# Autodesk Inventor assembly: Quadropod_assembly_v2
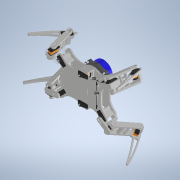
[picture p0: Inventor's stored thumbnail of the model, 180x180]
Saved by Autodesk Inventor 2020.3 (Build 243373000, 373)
## iProperties
Created: 2021-03-19
Part Number: Quadropod_assembly_v2
Document SubType Name: Assembly
Designer: sanyi
Author: sanyi
## Documents named in this file (15)
- C:\Users\sanyi\Documents\Inventor\Quadropod\Quadropod_assembly_v2.iam
- C:\Users\sanyi\Documents\Inventor\Quadropod\BaseBottom_v1.ipt
- C:\Users\sanyi\Documents\Inventor\Quadropod\LegPin_Middle_v1.ipt
- C:\Users\sanyi\Documents\Inventor\Quadropod\LegPin_Side_v1.ipt
- C:\Users\sanyi\Documents\Inventor\Quadropod\LegPin_Side_v1_MIR.ipt
- C:\Users\sanyi\Documents\Inventor\Quadropod\BaseTop_v1.ipt
- C:\Users\sanyi\Documents\Inventor\Quadropod\SH-0257MG.ipt
- C:\Users\sanyi\Documents\Inventor\Quadropod\LegStart_v1.ipt
- C:\Users\sanyi\Documents\Inventor\Quadropod\LegStart_v1_MIR.ipt
- C:\Users\sanyi\Documents\Inventor\Quadropod\ydlidar x4.ipt
- C:\Users\sanyi\Documents\Inventor\Quadropod\LegPin_v1.ipt
- C:\Users\sanyi\Documents\Inventor\Quadropod\LegMiddle_Final_1.ipt
- C:\Users\sanyi\Documents\Inventor\Quadropod\LegEnd_Right_v1.ipt
- C:\Users\sanyi\Documents\Inventor\Quadropod\LegEnd_Right_v1_MIR.ipt
- C:\Users\sanyi\Documents\Inventor\Quadropod\LegEnd_Right_v2.ipt
## Components (43 placed, 14 different names)
1. BaseBottom_v1:1 — Insert:1, Insert:2, Insert:3, Insert:4, Insert:5, Insert:6, Insert:7, Insert:8, Flush:1, Flush:2, Mate:1, Insert:9, Insert:10, Insert:11, Insert:12, Insert:15, Angle:1, Angle:2, Insert:16, Insert:17, Insert:18, Insert:19, Insert:20, Angle:3, Angle:4, Angle:5, Angle:6
2. LegPin_Middle_v1:1 — Insert:1, Insert:2
3. LegPin_Middle_v1:2 — Insert:3, Insert:4, Insert:13, Mate:2
4. LegPin_Middle_v1:3 — Insert:5, Insert:6
5. LegPin_Middle_v1:4 — Insert:7, Insert:8, Insert:14
6. LegPin_Side_v1:1 — Insert:9, Insert:10
7. LegPin_Side_v1_MIR:1 — Insert:11, Insert:12
8. BaseTop_v1:1 — Insert:13, Insert:14, Mate:2, Insert:59, Insert:60
9. SH-0257MG:1 — Insert:15, Angle:1, Insert:22
10. SH-0257MG:2 — Angle:2, Insert:16, Insert:23
11. SH-0257MG:3 — Insert:17, Angle:3
12. SH-0257MG:4 — Insert:20, Angle:6
13. SH-0257MG:5 — Insert:19, Angle:5, Insert:21
14. SH-0257MG:6 — Insert:18, Angle:4, Insert:24
15. LegStart_v1:2 — Insert:21, Insert:27, Angle:7, Insert:35, Insert:36
16. LegStart_v1:3 — Insert:23, Insert:30, Angle:10, Insert:31, Insert:32
17. LegStart_v1_MIR:1 — Insert:24, Insert:29, Angle:9, Insert:33, Insert:34
18. LegStart_v1_MIR:2 — Insert:22, Insert:28, Angle:8, Insert:37, Insert:38
19. ydlidar x4:1 — Flush:3, Insert:59, Insert:60
20. SH-0257MG:7 — Insert:27, Angle:7, Insert:41
21. SH-0257MG:8 — Insert:29, Angle:9, Insert:42
22. SH-0257MG:9 — Insert:28, Angle:8, Insert:39
23. SH-0257MG:10 — Insert:30, Angle:10, Insert:40
24. SH-0257MG:11 — Insert:55, Angle:15, Insert:63
25. SH-0257MG:12 — Insert:44, Angle:12, Insert:57
26. SH-0257MG:13 — Insert:45, Angle:13, Insert:58
27. SH-0257MG:14 — Insert:46, Angle:14, Insert:56
28. LegPin_v1:1 — Insert:31, Insert:32
29. LegPin_v1:2 — Insert:33, Insert:34
30. LegPin_v1:3 — Insert:37, Insert:38
31. LegPin_v1:4 — Insert:61, Insert:62
32. LegPin_v1:5 — Insert:49, Insert:50
33. LegPin_v1:6 — Insert:51, Insert:52
34. LegPin_v1:7 — Insert:53, Insert:54
35. LegPin_v1:8 — Insert:35, Insert:36
36. LegMiddle_Final_1:1 — Insert:39, Insert:56
37. LegMiddle_Final_1:2 — Insert:40, Insert:55
38. LegMiddle_Final_1:3 — Insert:42, Insert:58
39. LegMiddle_Final_1:4 — Insert:41, Insert:57
40. LegEnd_Right_v1:2 — Insert:44, Angle:12, Insert:49, Insert:50
41. LegEnd_Right_v1_MIR:1 — Insert:45, Angle:13, Insert:51, Insert:52
42. LegEnd_Right_v1_MIR:2 — Insert:46, Angle:14, Insert:53, Insert:54
43. LegEnd_Right_v2:1 — Angle:15, Insert:61, Insert:62, Insert:63
## Relationships (77: Insert 58, Angle 14, Flush 3, Mate 2)
- Insert:1: BaseBottom_v1:1 ↔ LegPin_Middle_v1:1
- Insert:2: BaseBottom_v1:1 ↔ LegPin_Middle_v1:1
- Insert:3: BaseBottom_v1:1 ↔ LegPin_Middle_v1:2
- Insert:4: BaseBottom_v1:1 ↔ LegPin_Middle_v1:2
- Insert:5: BaseBottom_v1:1 ↔ LegPin_Middle_v1:3
- Insert:6: BaseBottom_v1:1 ↔ LegPin_Middle_v1:3
- Insert:7: BaseBottom_v1:1 ↔ LegPin_Middle_v1:4
- Insert:8: BaseBottom_v1:1 ↔ LegPin_Middle_v1:4
- Flush:1: BaseBottom_v1:1
- Flush:2: BaseBottom_v1:1
- Mate:1: BaseBottom_v1:1
- Insert:9: BaseBottom_v1:1 ↔ LegPin_Side_v1:1
- Insert:10: BaseBottom_v1:1 ↔ LegPin_Side_v1:1
- Insert:11: BaseBottom_v1:1 ↔ LegPin_Side_v1_MIR:1
- Insert:12: BaseBottom_v1:1 ↔ LegPin_Side_v1_MIR:1
- Insert:13: LegPin_Middle_v1:2 ↔ BaseTop_v1:1
- Insert:14: LegPin_Middle_v1:4 ↔ BaseTop_v1:1
- Insert:15: BaseBottom_v1:1 ↔ SH-0257MG:1
- Angle:1 (0 deg): BaseBottom_v1:1 ↔ SH-0257MG:1
- Angle:2 (0 deg): BaseBottom_v1:1 ↔ SH-0257MG:2
- Insert:16: BaseBottom_v1:1 ↔ SH-0257MG:2
- Insert:17: BaseBottom_v1:1 ↔ SH-0257MG:3
- Insert:18: BaseBottom_v1:1 ↔ SH-0257MG:6
- Insert:19: BaseBottom_v1:1 ↔ SH-0257MG:5
- Insert:20: BaseBottom_v1:1 ↔ SH-0257MG:4
- Angle:3 (0 deg): BaseBottom_v1:1 ↔ SH-0257MG:3
- Angle:4 (0 deg): BaseBottom_v1:1 ↔ SH-0257MG:6
- Angle:5 (0 deg): BaseBottom_v1:1 ↔ SH-0257MG:5
- Angle:6 (0 deg): BaseBottom_v1:1 ↔ SH-0257MG:4
- Insert:21 (0.2 mm): SH-0257MG:5 ↔ LegStart_v1:2
- Insert:22 (0.2 mm): SH-0257MG:1 ↔ LegStart_v1_MIR:2
- Insert:23 (0.2 mm): SH-0257MG:2 ↔ LegStart_v1:3
- Insert:24 (0.2 mm): SH-0257MG:6 ↔ LegStart_v1_MIR:1
- Insert:27: LegStart_v1:2 ↔ SH-0257MG:7
- Angle:7 (0 deg): LegStart_v1:2 ↔ SH-0257MG:7
- Insert:28: LegStart_v1_MIR:2 ↔ SH-0257MG:9
- Angle:8 (0 deg): LegStart_v1_MIR:2 ↔ SH-0257MG:9
- Insert:29: LegStart_v1_MIR:1 ↔ SH-0257MG:8
- Angle:9 (0 deg): LegStart_v1_MIR:1 ↔ SH-0257MG:8
- Insert:30: LegStart_v1:3 ↔ SH-0257MG:10
- Angle:10 (0 deg): LegStart_v1:3 ↔ SH-0257MG:10
- Insert:31: LegStart_v1:3 ↔ LegPin_v1:1
- Insert:32: LegStart_v1:3 ↔ LegPin_v1:1
- Insert:33: LegStart_v1_MIR:1 ↔ LegPin_v1:2
- Insert:34: LegStart_v1_MIR:1 ↔ LegPin_v1:2
- Insert:35: LegStart_v1:2 ↔ LegPin_v1:8
- Insert:36: LegStart_v1:2 ↔ LegPin_v1:8
- Insert:37: LegStart_v1_MIR:2 ↔ LegPin_v1:3
- Insert:38: LegStart_v1_MIR:2 ↔ LegPin_v1:3
- Insert:39: SH-0257MG:9 ↔ LegMiddle_Final_1:1
- Insert:40: SH-0257MG:10 ↔ LegMiddle_Final_1:2
- Insert:41: SH-0257MG:7 ↔ LegMiddle_Final_1:4
- Insert:42: SH-0257MG:8 ↔ LegMiddle_Final_1:3
- Insert:44: SH-0257MG:12 ↔ LegEnd_Right_v1:2
- Insert:45: SH-0257MG:13 ↔ LegEnd_Right_v1_MIR:1
- Insert:46: SH-0257MG:14 ↔ LegEnd_Right_v1_MIR:2
- Angle:12 (0 deg): SH-0257MG:12 ↔ LegEnd_Right_v1:2
- Angle:13 (0 deg): SH-0257MG:13 ↔ LegEnd_Right_v1_MIR:1
- Angle:14 (0 deg): SH-0257MG:14 ↔ LegEnd_Right_v1_MIR:2
- Insert:49: LegPin_v1:5 ↔ LegEnd_Right_v1:2
- Insert:50: LegPin_v1:5 ↔ LegEnd_Right_v1:2
- Insert:51: LegPin_v1:6 ↔ LegEnd_Right_v1_MIR:1
- Insert:52: LegPin_v1:6 ↔ LegEnd_Right_v1_MIR:1
- Insert:53: LegPin_v1:7 ↔ LegEnd_Right_v1_MIR:2
- Insert:54: LegPin_v1:7 ↔ LegEnd_Right_v1_MIR:2
- Insert:55 (0.2 mm): SH-0257MG:11 ↔ LegMiddle_Final_1:2
- Insert:56 (0.2 mm): SH-0257MG:14 ↔ LegMiddle_Final_1:1
- Insert:57 (0.2 mm): SH-0257MG:12 ↔ LegMiddle_Final_1:4
- Insert:58 (0.2 mm): SH-0257MG:13 ↔ LegMiddle_Final_1:3
- Flush:3 (-9.4 mm): ydlidar x4:1
- Mate:2: LegPin_Middle_v1:2 ↔ BaseTop_v1:1
- Insert:59: BaseTop_v1:1 ↔ ydlidar x4:1
- Insert:60: BaseTop_v1:1 ↔ ydlidar x4:1
- Angle:15 (0 deg): SH-0257MG:11 ↔ LegEnd_Right_v2:1
- Insert:61: LegPin_v1:4 ↔ LegEnd_Right_v2:1
- Insert:62: LegPin_v1:4 ↔ LegEnd_Right_v2:1
- Insert:63: SH-0257MG:11 ↔ LegEnd_Right_v2:1
